# Autodesk Inventor assembly: Motors with Screws
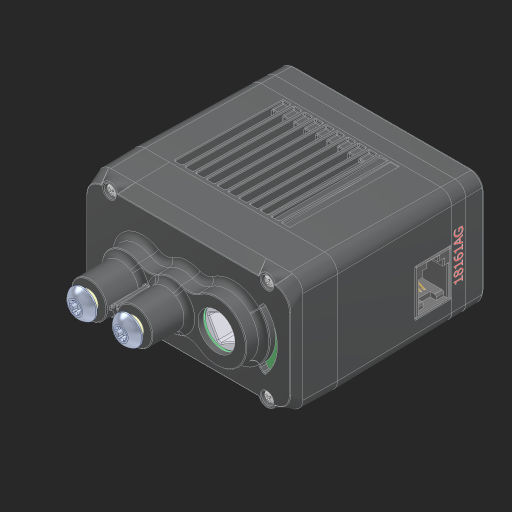
[picture p0: Inventor's stored thumbnail of the model, 512x512]
Saved by Autodesk Inventor 2023 (Build 270158000, 158)
## iProperties
Created: 2022-08-18
Part Number: Motors with Screws
Document SubType Name: Assembly
Designer: ylu12
Author: ylu12
## Documents named in this file (5)
- C:\Users\ylu12\Documents\GitHub\VEX-CAD-Inventor\Electronics\Motors with Screws\AluM-StarS.iam
- C:\Users\ylu12\Documents\GitHub\VEX-CAD-Inventor\Electronics\V5 Motor.ipt
- C:\Users\ylu12\Documents\GitHub\VEX-CAD-Inventor\Structure\Hardware\Screw Steel - Star\SScrew Star Smooth .500.ipt
- C:\Users\ylu12\Documents\GitHub\VEX-CAD-Inventor\Structure\Hardware\Screw Steel - Star.ipt
- C:\Users\ylu12\Documents\GitHub\VEX-CAD-Inventor\Electronics\Motors with Screws.iam
## Components (3 placed, 2 different names)
1. V5 Motor:1
2. SScrew Star Smooth .500:1
3. SScrew Star Smooth .500:2
## Named parameters: Thickness = 1.5875 mm
